# Autodesk Inventor assembly: Direccion
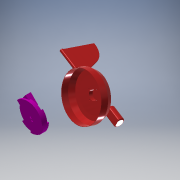
[picture p0: Inventor's stored thumbnail of the model, 180x180]
Saved by Autodesk Inventor 2019 (Build 230136000, 136)
## iProperties
Created: 2020-04-23
Part Number: Direccion
Document SubType Name: Assembly
Designer: Sergio
Author: Sergio
## Documents named in this file (4)
- C:\Users\Sergio\Documents\Innovandes\PROYECTO_GIT\EDITABLES\3D\VersionFinal\Viento\Direccion.iam
- C:\Users\Sergio\Documents\Innovandes\PROYECTO_GIT\EDITABLES\3D\Prototipo\3D\Modulos\Viento\DesnivelSharp.ipt
- C:\Users\Sergio\Documents\Innovandes\PROYECTO_GIT\EDITABLES\3D\Prototipo\3D\Modulos\Viento\DesnivelSharp2.ipt
- C:\Users\Sergio\Documents\Innovandes\PROYECTO_GIT\EDITABLES\3D\VersionFinal\Viento\Direccion.ipt
## Components (3 placed, 3 different names)
1. DesnivelSharp:1
2. DesnivelSharp2:1 — Mate:1, Mate:2
3. Direccion:1 — Mate:1, Mate:2
## Relationships (2: Mate 2)
- Mate:1: DesnivelSharp2:1 ↔ Direccion:1
- Mate:2: DesnivelSharp2:1 ↔ Direccion:1
